# Autodesk Inventor assembly: Sweeper Model
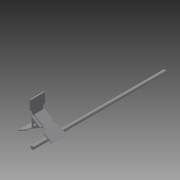
[picture p0: Inventor's stored thumbnail of the model, 180x180]
Saved by Autodesk Inventor 2014 (Build 180170000, 170)
## iProperties
Created: 2014-03-16
Part Number: Sweeper Model
Document SubType Name: Assembly
Designer: Pranav
Author: Pranav
## Documents named in this file (3)
- E:\Robotics Autodesk\Old Sweeper Model.iam
- E:\Robotics Autodesk\Sweeper Rod.ipt
- E:\Robotics Autodesk\Old Bush.iam
## Components (2 placed, 2 different names)
1. Sweeper Rod:1 — Rigid:1
2. Old Bush:1 [sub-assembly] — Rigid:1
## Relationships (1: WeldJoint 1)
- Rigid:1 [WeldJoint] (-10.16 mm): Sweeper Rod:1 ↔ Old Bush:1
